# Autodesk Inventor assembly: Gripper_Design_NonCompliant_No_UR5
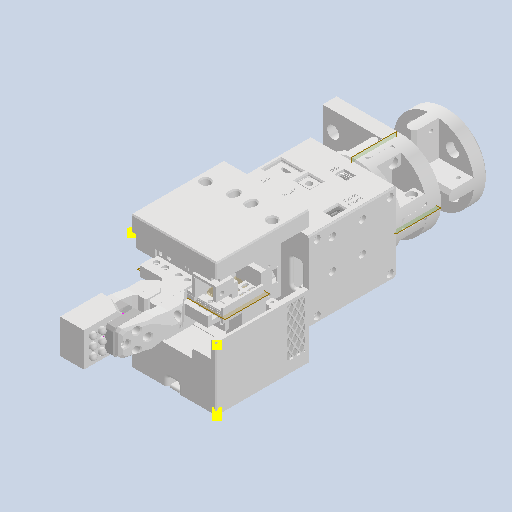
[picture p0: Inventor's stored thumbnail of the model, 512x512]
Saved by Autodesk Inventor 2022 (Build 260153000, 153)
## iProperties
Created: 2021-07-25
Part Number: Gripper_Design_NonCompliant_No_UR5
Document SubType Name: Assembly
Designer: exllu
Author: exllu
## Documents named in this file (30)
- C:\Users\kylem\OneDrive\Documents\GitHub\IMML_Contactile_Gripper_Hardware\Gripper_Design_NonCompliant_No_UR5.iam
- C:\Users\kylem\OneDrive\Documents\GitHub\IMML_Contactile_Gripper_Hardware\Motor_XM,H-430_idler.ipt
- C:\Users\kylem\OneDrive\Documents\GitHub\IMML_Contactile_Gripper_Hardware\Carriage_8381K550.iam
- C:\Users\kylem\OneDrive\Documents\GitHub\IMML_Contactile_Gripper_Hardware\Rail_8381K550.iam
- C:\Users\kylem\OneDrive\Documents\GitHub\IMML_Contactile_Gripper_Hardware\Pinion_2664N316.ipt
- C:\Users\kylem\OneDrive\Documents\GitHub\IMML_Contactile_Gripper_Hardware\Drive_shaft.ipt
- C:\Users\kylem\OneDrive\Documents\GitHub\IMML_Contactile_Gripper_Hardware\Motor_horn_mount.ipt
- C:\Users\kylem\OneDrive\Documents\GitHub\IMML_Contactile_Gripper_Hardware\Rack.iam
- C:\Users\kylem\OneDrive\Documents\GitHub\IMML_Contactile_Gripper_Hardware\Rail_lock_washer.ipt
- C:\Users\kylem\OneDrive\Documents\GitHub\IMML_Contactile_Gripper_Hardware\Rail_screws.ipt
- C:\Users\kylem\OneDrive\Documents\GitHub\IMML_Contactile_Gripper_Hardware\Rail_mount.ipt
- C:\Users\kylem\OneDrive\Documents\GitHub\IMML_Contactile_Gripper_Hardware\Front_plate.ipt
- C:\Users\kylem\OneDrive\Documents\GitHub\IMML_Contactile_Gripper_Hardware\Compliant_plate.ipt
- C:\Users\kylem\OneDrive\Documents\GitHub\IMML_Contactile_Gripper_Hardware\Padding.ipt
- C:\Users\kylem\OneDrive\Documents\GitHub\IMML_Contactile_Gripper_Hardware\UR5_Mounting_Plate.ipt
- C:\Users\kylem\OneDrive\Documents\GitHub\IMML_Contactile_Gripper_Hardware\Motor_UR5_mount.ipt
- C:\Users\kylem\OneDrive\Documents\GitHub\IMML_Contactile_Gripper_Hardware\Cover_bottom.ipt
- C:\Users\kylem\OneDrive\Documents\GitHub\IMML_Contactile_Gripper_Hardware\Cover_top.ipt
- C:\Users\kylem\OneDrive\Documents\GitHub\IMML_Contactile_Gripper_Hardware\Cover_bottom_raceway_cover.ipt
- C:\Users\kylem\OneDrive\Documents\GitHub\IMML_Contactile_Gripper_Hardware\U2D2 and Power Board Assembly.iam
- C:\Users\kylem\OneDrive\Documents\GitHub\IMML_Contactile_Gripper_Hardware\Contactile Communication Hub.ipt
- C:\Users\kylem\OneDrive\Documents\GitHub\IMML_Contactile_Gripper_Hardware\Electronics Box.ipt
- C:\Users\kylem\OneDrive\Documents\GitHub\IMML_Contactile_Gripper_Hardware\Electronics Box Lid.ipt
- C:\Users\kylem\OneDrive\Documents\GitHub\IMML_Contactile_Gripper_Hardware\Finger Assembly Left.iam
- C:\Users\kylem\OneDrive\Documents\GitHub\IMML_Contactile_Gripper_Hardware\Finger Assembly Right.iam
- C:\Users\kylem\OneDrive\Documents\GitHub\IMML_Contactile_Gripper_Hardware\IMU_assembly.iam
- C:\Users\kylem\OneDrive\Documents\GitHub\IMML_Contactile_Gripper_Hardware\Non_compliant_plate3.ipt
- C:\Users\kylem\OneDrive\Documents\GitHub\IMML_Contactile_Gripper_Hardware\Test_Stand_Mounting_Plate.ipt
- C:\Users\kylem\Downloads\Contactile_Controller.ipt
- C:\Users\kylem\Downloads\Contactile_Sensor.ipt
## Components (41 placed, 29 different names)
1. Motor_XM,H-430_idler:1 — Flush:1, Flush:2, Flush:3, Flush:7, Mate:15, Mate:16, Mate:29, Flush:22, Mate:65, Angle:2, Mate:223, Mate:226
2. Rail_8381K550:3 [sub-assembly] — Mate:3, Mate:4, Mate:5, Mate:6, Flush:7, Mate:29, Mate:30, Flush:18, Flush:19, Mate:40, Mate:41, Mate:44, Mate:45, Mate:47, Mate:55, Mate:56, Mate:57, Mate:59, Mate:61, Mate:62, Flush:25
3. Rail_8381K550:4 [sub-assembly] — Mate:1, Mate:2, Mate:7, Mate:8, Mate:30, Flush:18, Flush:19, Mate:46, Mate:63
4. Carriage_8381K550:5 [sub-assembly] — Mate:4, Mate:5, Flush:12, Flush:24, Mate:67, Mate:69
5. Carriage_8381K550:6 [sub-assembly] — Mate:1, Mate:7
6. Carriage_8381K550:7 [sub-assembly] — Mate:3, Mate:6, Mate:262, Mate:263, Mate:264
7. Carriage_8381K550:8 [sub-assembly] — Mate:2, Mate:8, Flush:23, Mate:277
8. Pinion_2664N316:1 — Mate:20, Mate:21, Flush:20, Tangent:1, Tangent:2, Rotation/Translation:1
9. Drive_shaft:1 — Mate:17, Mate:20, Mate:21, Mate:66, Mate:228
10. Motor_horn_mount:1 — Mate:15, Mate:16, Mate:17, Mate:64, Mate:66, Mate:227, Mate:228
11. Rack:1 [sub-assembly] — Flush:20, Tangent:1, Flush:23, Mate:276
12. Rack:2 [sub-assembly] — Flush:12, Tangent:2, Rotation/Translation:1, Mate:70
13. Rail_lock_washer:1 — Mate:40, Mate:41
14. Rail_lock_washer:3 — Mate:44, Mate:47, Mate:54
15. Rail_lock_washer:4 — Mate:45, Mate:46, Mate:60
16. Rail_screws:1 — Mate:60, Mate:61
17. Rail_screws:2 — Mate:54, Mate:55
18. Rail_screws:3 — Mate:58, Mate:59
19. Rail_lock_washer:5 — Mate:56, Mate:57, Mate:58
20. Rail_mount:1 — Mate:62, Mate:63, Flush:25, Mate:68, Mate:135
21. Front_plate:1 — Flush:22, Mate:64, Mate:65, Mate:68, Mate:227
22. Compliant_plate:1 — Flush:24, Mate:67, Mate:69, Mate:70, Mate:139
23. Padding:1 — Mate:139
24. UR5_Mounting_Plate:1 — Mate:129
25. Motor_UR5_mount:1 — Mate:129, Mate:254, Mate:256, Mate:258, Mate:268, Mate:269
26. Cover_bottom:1 — Mate:135, Flush:35, Mate:142, Mate:143, Flush:50, Mate:225, Mate:261
27. Cover_top:1 — Flush:35, Mate:224
28. Cover_bottom_raceway_cover:1 — Mate:142, Mate:143, Mate:261
29. U2D2 and Power Board Assembly:1 [sub-assembly] — Angle:2, Flush:49, Mate:216, Mate:218, Flush:51
30. Contactile Communication Hub:1 — Flush:49, Mate:220
31. Electronics Box:1 — Flush:50, Mate:216, Mate:218, Mate:219, Mate:220, Mate:223, Mate:224, Mate:225, Mate:226, Flush:51, Mate:251, Mate:253, Mate:254, Mate:255, Mate:256, Mate:258, Mate:270, Flush:55, Mate:273, Mate:274
32. Electronics Box Lid:1 — Mate:219, Mate:270
33. Finger Assembly Right:1 [sub-assembly] — Mate:278, Flush:57, Flush:58, Mate:279
34. Finger Assembly Left:1 [sub-assembly] — Flush:54, Mate:266, Mate:275, Flush:56
35. IMU_assembly:1 [sub-assembly] — Mate:251, Mate:253, Mate:255
36. Non_compliant_plate3:1 — Mate:262, Mate:263, Mate:264, Flush:54, Mate:266, Flush:56, Mate:281, Flush:60
37. Test_Stand_Mounting_Plate:1 — Mate:268, Mate:269
38. Contactile_Controller:1 — Flush:55, Mate:273, Mate:274
39. Contactile_Sensor:1 — Mate:279, Mate:280, Flush:59
40. Contactile_Sensor:2 — Mate:275, Mate:281, Flush:60
41. Non_compliant_plate3:2 — Mate:276, Mate:277, Mate:278, Flush:57, Flush:58, Mate:280, Flush:59
## Relationships (103: Mate 76, Flush 23, Tangent 2, RelateRotateTranslate 1, Angle 1)
- Mate:1 (0.1 mm): Rail_8381K550:4 ↔ Carriage_8381K550:6
- Mate:2 (0.1 mm): Rail_8381K550:4 ↔ Carriage_8381K550:8
- Mate:3 (0.1 mm): Rail_8381K550:3 ↔ Carriage_8381K550:7
- Mate:4 (0.1 mm): Rail_8381K550:3 ↔ Carriage_8381K550:5
- Mate:5 (0.2 mm): Rail_8381K550:3 ↔ Carriage_8381K550:5
- Mate:6 (0.2 mm): Rail_8381K550:3 ↔ Carriage_8381K550:7
- Mate:7 (0.2 mm): Rail_8381K550:4 ↔ Carriage_8381K550:6
- Mate:8 (0.2 mm): Rail_8381K550:4 ↔ Carriage_8381K550:8
- Flush:1: Motor_XM,H-430_idler:1
- Flush:2: Motor_XM,H-430_idler:1
- Flush:3: Motor_XM,H-430_idler:1
- Flush:7 (-20.75 mm): Motor_XM,H-430_idler:1 ↔ Rail_8381K550:3
- Mate:15: Motor_XM,H-430_idler:1 ↔ Motor_horn_mount:1
- Mate:16: Motor_XM,H-430_idler:1 ↔ Motor_horn_mount:1
- Mate:17: Drive_shaft:1 ↔ Motor_horn_mount:1
- Mate:20: Pinion_2664N316:1 ↔ Drive_shaft:1
- Mate:21: Pinion_2664N316:1 ↔ Drive_shaft:1
- Flush:12: Carriage_8381K550:5 ↔ Rack:2
- Mate:29 (-10.75 mm): Motor_XM,H-430_idler:1 ↔ Rail_8381K550:3
- Mate:30 (1 mm): Rail_8381K550:3 ↔ Rail_8381K550:4
- Flush:18: Rail_8381K550:3 ↔ Rail_8381K550:4
- Flush:19: Rail_8381K550:3 ↔ Rail_8381K550:4
- Flush:20: Pinion_2664N316:1 ↔ Rack:1
- Mate:40: Rail_8381K550:3 ↔ Rail_lock_washer:1
- Mate:41: Rail_8381K550:3 ↔ Rail_lock_washer:1
- Mate:44: Rail_8381K550:3 ↔ Rail_lock_washer:3
- Mate:45: Rail_8381K550:3 ↔ Rail_lock_washer:4
- Mate:46: Rail_8381K550:4 ↔ Rail_lock_washer:4
- Mate:47: Rail_8381K550:3 ↔ Rail_lock_washer:3
- Mate:54: Rail_lock_washer:3 ↔ Rail_screws:2
- Mate:55: Rail_8381K550:3 ↔ Rail_screws:2
- Mate:56: Rail_8381K550:3 ↔ Rail_lock_washer:5
- Mate:57: Rail_8381K550:3 ↔ Rail_lock_washer:5
- Mate:58: Rail_screws:3 ↔ Rail_lock_washer:5
- Mate:59: Rail_8381K550:3 ↔ Rail_screws:3
- Mate:60: Rail_lock_washer:4 ↔ Rail_screws:1
- Mate:61: Rail_8381K550:3 ↔ Rail_screws:1
- Mate:62: Rail_8381K550:3 ↔ Rail_mount:1
- Mate:63: Rail_8381K550:4 ↔ Rail_mount:1
- Flush:22: Motor_XM,H-430_idler:1 ↔ Front_plate:1
- Mate:64: Motor_horn_mount:1 ↔ Front_plate:1
- Mate:65: Motor_XM,H-430_idler:1 ↔ Front_plate:1
- Tangent:1 (-1 mm): Pinion_2664N316:1 ↔ Rack:1
- Tangent:2 (-1 mm): Pinion_2664N316:1 ↔ Rack:2
- Rotation/Translation:1 [RelateRotateTranslate] (39.841 mm): Pinion_2664N316:1 ↔ Rack:2
- Mate:66: Drive_shaft:1 ↔ Motor_horn_mount:1
- Flush:23: Carriage_8381K550:8 ↔ Rack:1
- Flush:24: Carriage_8381K550:5 ↔ Compliant_plate:1
- Mate:67: Carriage_8381K550:5 ↔ Compliant_plate:1
- Flush:25: Rail_8381K550:3 ↔ Rail_mount:1
- Mate:68: Rail_mount:1 ↔ Front_plate:1
- Mate:69: Carriage_8381K550:5 ↔ Compliant_plate:1
- Mate:70: Rack:2 ↔ Compliant_plate:1
- Mate:129: UR5_Mounting_Plate:1 ↔ Motor_UR5_mount:1
- Mate:135 (0.5 mm): Rail_mount:1 ↔ Cover_bottom:1
- Mate:139: Compliant_plate:1 ↔ Padding:1
- Flush:35: Cover_bottom:1 ↔ Cover_top:1
- Mate:142: Cover_bottom:1 ↔ Cover_bottom_raceway_cover:1
- Mate:143: Cover_bottom:1 ↔ Cover_bottom_raceway_cover:1
- Angle:2 (180 deg): Motor_XM,H-430_idler:1 ↔ U2D2 and Power Board Assembly:1
- Flush:49 (-1 mm): U2D2 and Power Board Assembly:1 ↔ Contactile Communication Hub:1
- Flush:50: Cover_bottom:1 ↔ Electronics Box:1
- Mate:216 (9 mm): U2D2 and Power Board Assembly:1 ↔ Electronics Box:1
- Mate:218 (1 mm): U2D2 and Power Board Assembly:1 ↔ Electronics Box:1
- Mate:219: Electronics Box:1 ↔ Electronics Box Lid:1
- Mate:220 (1 mm): Contactile Communication Hub:1 ↔ Electronics Box:1
- Mate:223: Motor_XM,H-430_idler:1 ↔ Electronics Box:1
- Mate:224: Cover_top:1 ↔ Electronics Box:1
- Mate:225: Cover_bottom:1 ↔ Electronics Box:1
- Mate:226: Motor_XM,H-430_idler:1 ↔ Electronics Box:1
- Flush:51 (2 mm): U2D2 and Power Board Assembly:1 ↔ Electronics Box:1
- Mate:227: Motor_horn_mount:1 ↔ Front_plate:1
- Mate:228: Drive_shaft:1 ↔ Motor_horn_mount:1
- Mate:251: Electronics Box:1 ↔ IMU_assembly:1
- Mate:253: Electronics Box:1 ↔ IMU_assembly:1
- Mate:254: Motor_UR5_mount:1 ↔ Electronics Box:1
- Mate:255: Electronics Box:1 ↔ IMU_assembly:1
- Mate:256: Motor_UR5_mount:1 ↔ Electronics Box:1
- Mate:258: Motor_UR5_mount:1 ↔ Electronics Box:1
- Mate:261 (0.5 mm): Cover_bottom:1 ↔ Cover_bottom_raceway_cover:1
- Mate:262: Carriage_8381K550:7 ↔ Non_compliant_plate3:1
- Mate:263: Carriage_8381K550:7 ↔ Non_compliant_plate3:1
- Mate:264: Carriage_8381K550:7 ↔ Non_compliant_plate3:1
- Flush:54: Finger Assembly Left:1 ↔ Non_compliant_plate3:1
- Mate:266: Finger Assembly Left:1 ↔ Non_compliant_plate3:1
- Mate:268: Motor_UR5_mount:1 ↔ Test_Stand_Mounting_Plate:1
- Mate:269: Motor_UR5_mount:1 ↔ Test_Stand_Mounting_Plate:1
- Mate:270: Electronics Box:1 ↔ Electronics Box Lid:1
- Flush:55 (3 mm): Electronics Box:1 ↔ Contactile_Controller:1
- Mate:273: Electronics Box:1 ↔ Contactile_Controller:1
- Mate:274 (14 mm): Electronics Box:1 ↔ Contactile_Controller:1
- Mate:275: Finger Assembly Left:1 ↔ Contactile_Sensor:2
- Flush:56: Finger Assembly Left:1 ↔ Non_compliant_plate3:1
- Mate:276: Rack:1 ↔ Non_compliant_plate3:2
- Mate:277: Carriage_8381K550:8 ↔ Non_compliant_plate3:2
- Mate:278: Finger Assembly Right:1 ↔ Non_compliant_plate3:2
- Flush:57: Finger Assembly Right:1 ↔ Non_compliant_plate3:2
- Flush:58: Finger Assembly Right:1 ↔ Non_compliant_plate3:2
- Mate:279: Finger Assembly Right:1 ↔ Contactile_Sensor:1
- Mate:280 (11 mm): Contactile_Sensor:1 ↔ Non_compliant_plate3:2
- Mate:281 (11 mm): Non_compliant_plate3:1 ↔ Contactile_Sensor:2
- Flush:59 (-2.5 mm): Contactile_Sensor:1 ↔ Non_compliant_plate3:2
- Flush:60 (-2.5 mm): Non_compliant_plate3:1 ↔ Contactile_Sensor:2
